# Autodesk Inventor assembly: Palm
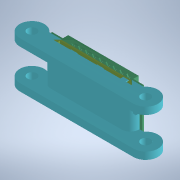
[picture p0: Inventor's stored thumbnail of the model, 180x180]
Saved by Autodesk Inventor 2020 (Build 240168000, 168)
## iProperties
Created: 2019-10-21
Part Number: Palm
Document SubType Name: Assembly
Designer: ayad493
Author: ayad493
## Documents named in this file (4)
- \\files.auckland.ac.nz\myhome\Downloads\MECHENG730\Project3\CAD\ModularFinger\Palm.iam
- \\files.auckland.ac.nz\myhome\Downloads\MECHENG730\Project3\CAD\ModularFinger\mPalm.ipt
- \\files.auckland.ac.nz\myhome\Downloads\MECHENG730\Project3\CAD\ModularFinger\PalmSupport.ipt
- \\files.auckland.ac.nz\myhome\Downloads\MECHENG730\Project3\CAD\ModularFinger\Palm_Grip.ipt
## Components (3 placed, 3 different names)
1. mPalm:1 — Mate:1, Mate:2, Mate:3, Mate:4
2. PalmSupport:1 — Mate:1
3. Palm_Grip:1 — Mate:2, Mate:3, Mate:4
## Relationships (4: Mate 4)
- Mate:1: mPalm:1 ↔ PalmSupport:1
- Mate:2: mPalm:1 ↔ Palm_Grip:1
- Mate:3: mPalm:1 ↔ Palm_Grip:1
- Mate:4: mPalm:1 ↔ Palm_Grip:1
